# Autodesk Inventor assembly: Final_Head
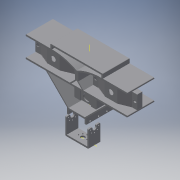
[picture p0: Inventor's stored thumbnail of the model, 180x180]
Saved by Autodesk Inventor 2016 (Build 200138000, 138)
## iProperties
Created: 2015-09-28
Part Number: Final_Head
Document SubType Name: Assembly
Designer: fei
Author: fei
## Documents named in this file (5)
- C:\Users\fei\Desktop\Robot_Head\Final_Head.iam
- C:\Users\fei\Desktop\Robot_Head\Test2.ipt
- C:\Users\fei\Desktop\Robot_Head\Camera.iam
- C:\Users\fei\Desktop\Robot_Head\Down_Part_Robot.ipt
- C:\Users\fei\Desktop\Robot_Head\Speaker.ipt
## Components (5 placed, 4 different names)
1. Test2:1 — Insert:1, Insert:2, Insert:3
2. Camera:1 [sub-assembly] — Insert:1
3. Camera:2 [sub-assembly] — Insert:2
4. Down_Part_Robot:1
5. Speaker:1 — Insert:3
## Relationships (3: Insert 3)
- Insert:1: Test2:1 ↔ Camera:1
- Insert:2: Test2:1 ↔ Camera:2
- Insert:3: Test2:1 ↔ Speaker:1
